# Autodesk Inventor assembly: OLED_With_Carrier
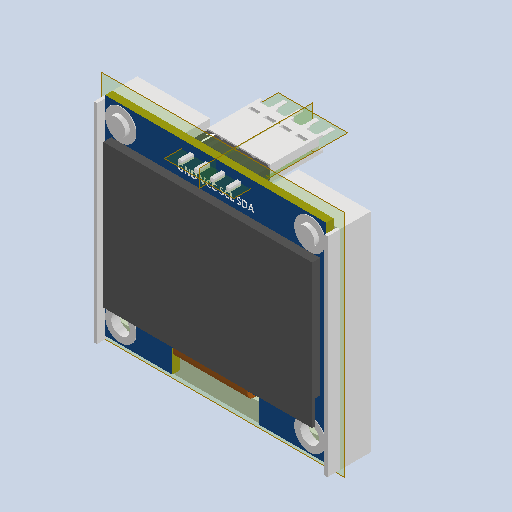
[picture p0: Inventor's stored thumbnail of the model, 512x512]
Saved by Autodesk Inventor 2024.3 (Build 283343000, 343)
## iProperties
Created: 2024-05-11
Part Number: OLED_With_Carrier
Document SubType Name: Assembly
Designer: atrus
Author: atrus
## Documents named in this file (3)
- C:\Users\atrus\Dropbox\elec\Mechanical\DCBuddyV2\OLED_With_Carrier.iam
- C:\Users\atrus\Dropbox\elec\Mechanical\DCBuddyV2\User Library-OLED-1_3-128X64.iam
- C:\Users\atrus\Dropbox\elec\Mechanical\DCBuddyV2\OledCarrier.ipt
## Components (2 placed, 2 different names)
1. User Library-OLED-1_3-128X64:1 [sub-assembly] — Flush:1, Flush:2
2. OledCarrier:1 — Flush:1, Flush:2
## Relationships (2: Flush 2)
- Flush:1: User Library-OLED-1_3-128X64:1 ↔ OledCarrier:1
- Flush:2: User Library-OLED-1_3-128X64:1 ↔ OledCarrier:1
